# Autodesk Inventor assembly: TBeam
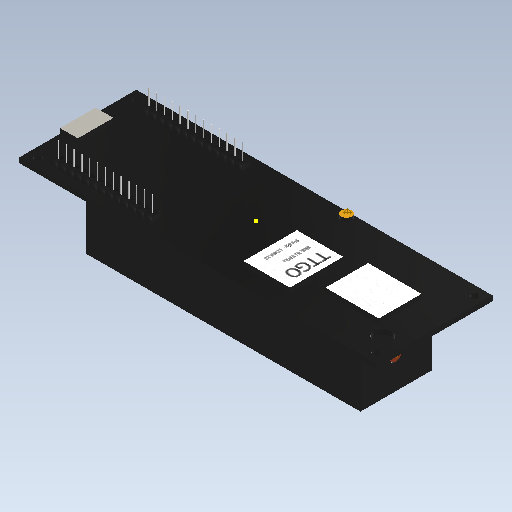
[picture p0: Inventor's stored thumbnail of the model, 512x512]
Saved by Autodesk Inventor 2020 (Build 240168000, 168)
## iProperties
Created: 2022-02-21
Part Number: TBeam
Document SubType Name: Assembly
Designer: DANIEL
Author: DANIEL
## Documents named in this file (4)
- C:\Users\DANIEL\Documents\Personal\Convocatorias\Escollera\tesis\CAD\V3\TBeam.iam
- C:\Users\DANIEL\Documents\Personal\Convocatorias\Escollera\tesis\CAD\V3\PlacaTBeam.ipt
- C:\Users\DANIEL\Documents\Personal\Convocatorias\Escollera\tesis\CAD\V3\patasTBeam.iam
- C:\Users\DANIEL\Documents\Personal\Convocatorias\Escollera\tesis\CAD\V3\portapilasIndividual.ipt
## Components (4 placed, 3 different names)
1. PlacaTBeam:1 — Coincidencia:1, Coincidencia:2, Coincidencia:3, Coincidencia:4, Coincidencia:5
2. patasTBeam:1 [sub-assembly] — Coincidencia:3, Coincidencia:4
3. patasTBeam:2 [sub-assembly] — Coincidencia:1, Coincidencia:2
4. portapilasIndividual:1 — Coincidencia:5
## Relationships (5: Mate 5)
- Coincidencia:1 [Mate] (6.13 mm): PlacaTBeam:1 ↔ patasTBeam:2
- Coincidencia:2 [Mate] (-5 mm): PlacaTBeam:1 ↔ patasTBeam:2
- Coincidencia:3 [Mate] (6.13 mm): PlacaTBeam:1 ↔ patasTBeam:1
- Coincidencia:4 [Mate] (-5 mm): PlacaTBeam:1 ↔ patasTBeam:1
- Coincidencia:5 [Mate]: PlacaTBeam:1 ↔ portapilasIndividual:1
